# Autodesk Inventor assembly: Toaster with middle air layer
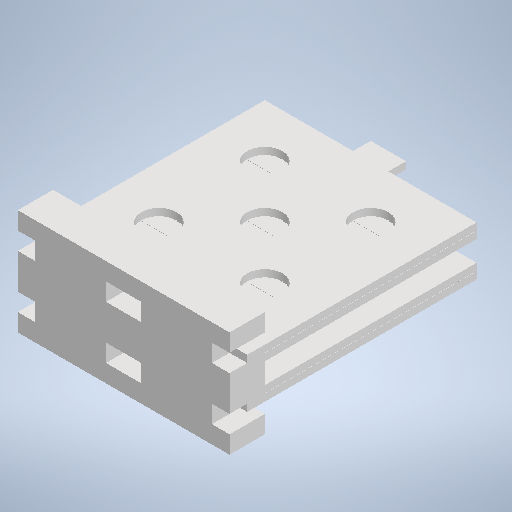
[picture p0: Inventor's stored thumbnail of the model, 512x512]
Saved by Autodesk Inventor 2025.1 (Build 291241020, 241B)
## iProperties
Created: 2024-10-29
Part Number: Toaster with middle air layer
Document SubType Name: Assembly
Designer: jjk
Author: jjk
## Documents named in this file (4)
- C:\Users\jjk\Desktop\Capstone CAD\Version 2\Toaster with middle air layer.iam
- C:\Users\jjk\Desktop\Capstone CAD\Version 3\Base.ipt
- C:\Users\jjk\Desktop\Capstone CAD\Version 3\Heating plate with 11 heating wires.iam
- C:\Users\jjk\Desktop\Capstone CAD\Version 3\air layer.ipt
## Components (5 placed, 3 different names)
1. Base:1 — Mate:1, Mate:2, Flush:1, Mate:3, Mate:4, Flush:2, Mate:5, Flush:7, Mate:7
2. Heating plate with 11 heating wires:1 [sub-assembly] — Mate:1, Mate:2, Flush:1, Mate:6
3. Heating plate with 11 heating wires:2 [sub-assembly] — Mate:3, Mate:4, Flush:2, Flush:8, Mate:8
4. air layer:1 — Mate:5, Flush:7, Mate:6
5. air layer:2 — Flush:8, Mate:7, Mate:8
## Relationships (12: Mate 8, Flush 4)
- Mate:1: Base:1 ↔ Heating plate with 11 heating wires:1
- Mate:2: Base:1 ↔ Heating plate with 11 heating wires:1
- Flush:1: Base:1 ↔ Heating plate with 11 heating wires:1
- Mate:3: Base:1 ↔ Heating plate with 11 heating wires:2
- Mate:4: Base:1 ↔ Heating plate with 11 heating wires:2
- Flush:2: Base:1 ↔ Heating plate with 11 heating wires:2
- Mate:5: Base:1 ↔ air layer:1
- Flush:7: Base:1 ↔ air layer:1
- Mate:6 (0.2032 mm): Heating plate with 11 heating wires:1 ↔ air layer:1
- Flush:8: Heating plate with 11 heating wires:2 ↔ air layer:2
- Mate:7: Base:1 ↔ air layer:2
- Mate:8 (0.2032 mm): Heating plate with 11 heating wires:2 ↔ air layer:2
